# Autodesk Inventor assembly: basketservoback
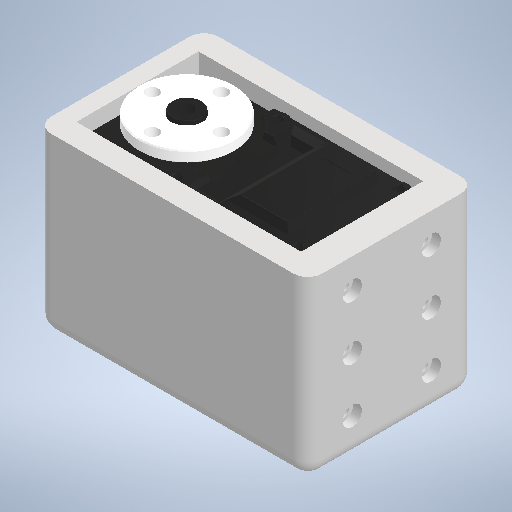
[picture p0: Inventor's stored thumbnail of the model, 512x512]
Saved by Autodesk Inventor 2025.3 (Build 293356000, 356)
## iProperties
Created: 2026-04-12
Part Number: basketservoback
Document SubType Name: Assembly
Designer: ksawe
Author: ksawe
## Documents named in this file (3)
- C:\Users\ksawe\OneDrive\Pulpit\Exomy v1\wersja2\basketservoback.iam
- C:\Users\ksawe\OneDrive\Pulpit\Exomy v1\wersja2\basketback.ipt
- C:\Users\ksawe\OneDrive\Pulpit\Exomy v1\wersja2\ST3215\ST3215\ST3215.ipt
## Components (2 placed, 2 different names)
1. basketback:1 — Mate:1, Mate:2, Mate:3
2. ST3215:1 — Mate:1, Mate:2, Mate:3
## Relationships (3: Mate 3)
- Mate:1: basketback:1 ↔ ST3215:1
- Mate:2: basketback:1 ↔ ST3215:1
- Mate:3: basketback:1 ↔ ST3215:1
